# Autodesk Inventor assembly: botAssemblyVer3
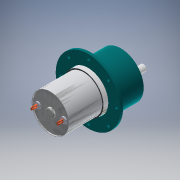
[picture p0: Inventor's stored thumbnail of the model, 180x180]
Saved by Autodesk Inventor 2016 (Build 200138000, 138)
## iProperties
Created: 2016-06-30
Part Number: botAssemblyVer3
Document SubType Name: Assembly
Designer: hesaon
Author: hesaon
## Documents named in this file (3)
- C:\Users\hesaon\Documents\Killer-Bot-2016\AutodeskWorkspace\robot parts revision 3\botAssemblyVer3.iam
- C:\Users\hesaon\Documents\Killer-Bot-2016\AutodeskWorkspace\robot parts revision 3\motor fixture.ipt
- C:\Users\hesaon\Documents\Killer-Bot-2016\AutodeskWorkspace\robotparts revision 2\37D mm metal gearmotor.ipt
## Components (2 placed, 2 different names)
1. motor fixture:1 — Insert:1, Insert:2
2. 37D mm metal gearmotor:1 — Insert:1, Insert:2
## Relationships (2: Insert 2)
- Insert:1: motor fixture:1 ↔ 37D mm metal gearmotor:1
- Insert:2: motor fixture:1 ↔ 37D mm metal gearmotor:1
